# Autodesk Inventor assembly: gear-sub
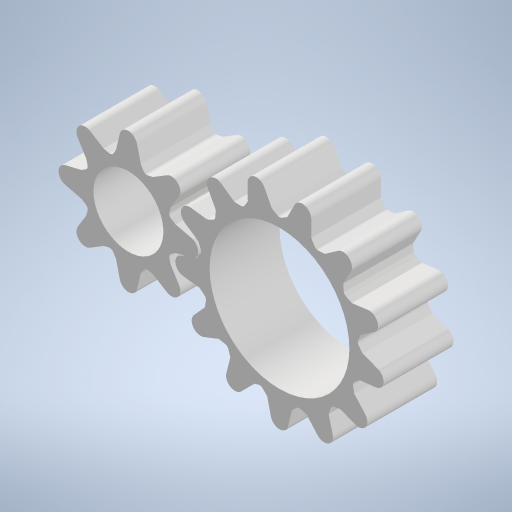
[picture p0: Inventor's stored thumbnail of the model, 512x512]
Saved by Autodesk Inventor 2023.2 (Build 272271000, 271)
## iProperties
Created: 2023-03-04
Part Number: gear-sub
Document SubType Name: Assembly
Designer: sarp1
Author: sarp1
## Documents named in this file (5)
- C:\Users\sarp1\Documents\hudson2022\gear-sub.iam
- C:\Users\sarp1\Documents\hudson2022\gear-sub\Design Accelerator\Spur Gears1.iam
- C:\Users\sarp1\Documents\hudson2022\gear-sub\Design Accelerator\Spur Gears2.iam
- C:\Users\sarp1\Documents\hudson2022\gearsub-hm.ipt
- C:\Users\sarp1\Documents\hudson2022\gearsub-hm2.ipt
## Components (4 placed, 3 different names)
1. Spur Gears:1 [sub-assembly]
2. Spur Gears:2 [sub-assembly]
3. gearsub-hm:1 — Mate:1, Rotation:1
4. gearsub-hm2:1 — Mate:2, Rotation:1
## Relationships (3: Mate 2, RelateRotation 1)
- Mate:1: gearsub-hm:1
- Mate:2: gearsub-hm2:1
- Rotation:1 [RelateRotation] (3 ul): gearsub-hm:1 ↔ gearsub-hm2:1
